# Autodesk Inventor assembly: Baugruppe1
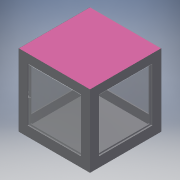
[picture p0: Inventor's stored thumbnail of the model, 180x180]
Saved by Autodesk Inventor 2018.3 (Build 223284000, 284)
## iProperties
Created: 2019-09-20
Part Number: Baugruppe1
Material: Generisch
Document SubType Name: Assembly
Designer: Lolob
Author: Lolob
Title: SmartCube
## Documents named in this file (6)
- D:\Dokumente\S ch u l e\Dipl\Smartcube_Construction\Version_3\Baugruppe1.iam
- D:\Dokumente\S ch u l e\Dipl\Smartcube_Construction\Version_2\PV_Modul_CPY_3.ipt
- D:\Dokumente\S ch u l e\Dipl\Smartcube_Construction\Version_3\Boden.ipt
- D:\Dokumente\S ch u l e\Dipl\Smartcube_Construction\Version_3\Boden_2.ipt
- D:\Dokumente\S ch u l e\Dipl\Smartcube_Construction\Version_3\PV_Rahmen.ipt
- D:\Dokumente\S ch u l e\Dipl\Smartcube_Construction\Version_2\PV_Modul.ipt
## Components (10 placed, 5 different names)
1. Sitzfläche:1 — Starr:2
2. PV_Modul_CPY_3:1 — Starr:1
3. Boden_2:1 — Starr:3
4. PV_Rahmen:1 — Starr:1, Starr:2, Starr:3, Starr:4
5. PV_Rahmen:2 — Starr:4, Starr:5, Drehbar:1
6. PV_Rahmen:3 — Starr:5, Starr:6, Starr:8
7. PV_Rahmen:4 — Starr:6, Starr:7
8. PV_Modul:1 — Starr:7
9. PV_Modul:2 — Drehbar:1
10. PV_Modul:3 — Starr:8
## Relationships (9: WeldJoint 8, RevoluteJoint 1)
- Starr:1 [WeldJoint]: PV_Modul_CPY_3:1 ↔ PV_Rahmen:1
- Starr:2 [WeldJoint]: Sitzfläche:1 ↔ PV_Rahmen:1
- Starr:3 [WeldJoint]: Boden_2:1 ↔ PV_Rahmen:1
- Starr:4 [WeldJoint]: PV_Rahmen:1 ↔ PV_Rahmen:2
- Starr:5 [WeldJoint]: PV_Rahmen:2 ↔ PV_Rahmen:3
- Starr:6 [WeldJoint]: PV_Rahmen:3 ↔ PV_Rahmen:4
- Starr:7 [WeldJoint] (3 mm): PV_Rahmen:4 ↔ PV_Modul:1
- Starr:8 [WeldJoint] (3 mm): PV_Rahmen:3 ↔ PV_Modul:3
- Drehbar:1 [RevoluteJoint]: PV_Rahmen:2 ↔ PV_Modul:2
